# Autodesk Inventor assembly: item_0043746_automatik-verbindungssatz_5_details_3
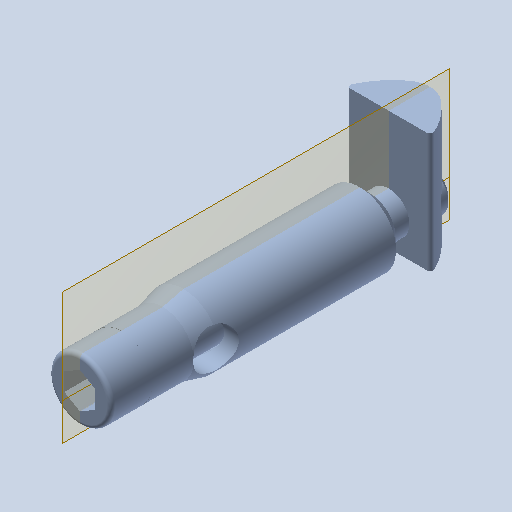
[picture p0: Inventor's stored thumbnail of the model, 512x512]
Saved by Autodesk Inventor 2024 (Build 280153000, 153)
## iProperties
Company: TraceParts S.A.
Created: 2022-11-13
Part Number: item_0043746_automatik-verbindungssatz_5_details_3
Checked By: TraceParts S.A.
Catalog Web Link: www.traceparts.com
Document SubType Name: Assembly
Designer: TraceParts
REFERENCE: 0.0.437.46
SELECTION: 0.0.437.46
SUPPLIER: item Industrietechnik GmbH
DESIGN: Automatik-Verbindungssatz 5, rostfrei
TraceParts.PartNumber: 30-12112020-080552
TraceParts.PartTitle: Automatik-Verbindungssatz 5, rostfrei
TraceParts.InstanceId: 30-12112020-0805526CLQ1VNJK2SV4842NLIXTZCD6
TRACEPARTS: TRACEPARTS
TraceParts.PartLanguage: de
TraceParts.PartVersion: 1.0.6
Author: TraceParts
## Documents named in this file (4)
- C:\Users\AEWALDER\Documents\Inventor\03_CurrentProjects\MasterThesis\PSM_V1_Rillenkugellager\Maschinenbauteil\item_0043746_automatik-verbindungssatz_5_details_3.iam
- C:\Users\AEWALDER\Documents\Inventor\03_CurrentProjects\MasterThesis\PSM_V1_Rillenkugellager\Maschinenbauteil\item_0043746_automatik-verbindungssatz_5_details_3_01.ipt
- C:\Users\AEWALDER\Documents\Inventor\03_CurrentProjects\MasterThesis\PSM_V1_Rillenkugellager\Maschinenbauteil\item_0043746_automatik-verbindungssatz_5_details_3_02.ipt
- C:\Users\AEWALDER\Documents\Inventor\03_CurrentProjects\MasterThesis\PSM_V1_Rillenkugellager\Maschinenbauteil\item_0043746_automatik-verbindungssatz_5_details_3_03.ipt
## Components (3 placed, 3 different names)
1. item_0043746_automatik-verbindungssatz_5_details_3_01:1
2. item_0043746_automatik-verbindungssatz_5_details_3_02:1 — Passend:1
3. item_0043746_automatik-verbindungssatz_5_details_3_03:1
## Relationships (2: Mate 1, Flush 1)
- Passend:1 [Mate]: item_0043746_automatik-verbindungssatz_5_details_3_02:1
- Fluchtend:1 [Flush]
